# Autodesk Inventor assembly: Lift Assembly
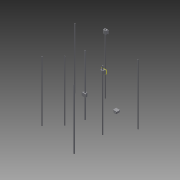
[picture p0: Inventor's stored thumbnail of the model, 180x180]
Saved by Autodesk Inventor 2013 (Build 170138000, 138)
## iProperties
Created: 2013-01-16
Part Number: Lift Assembly
Document SubType Name: Assembly
Designer: actoennies
Author: actoennies
## Documents named in this file (3)
- \\NNHSSRV2.hs.sd203.org\ACToennies$\Robotics\Lift\Lift Assembly.iam
- \\NNHSSRV2.hs.sd203.org\ACToennies$\Robotics\Lift\Tube.ipt
- \\NNHSSRV2.hs.sd203.org\ACToennies$\Inventor\Linear Bearing.ipt
## Components (12 placed, 2 different names)
1. Tube:1 — Mate:6, Mate:7
2. Tube:2 — Mate:1, Mate:2
3. Tube:3
4. Tube:4 — Mate:4, Mate:5
5. Tube:5
6. Tube:6
7. Tube:7
8. Tube:8
9. Linear Bearing:1 — Mate:1, Mate:2, Mate:3, Angle:1
10. Linear Bearing:2 — Mate:4, Mate:5
11. Linear Bearing:3 — Mate:6, Mate:7
12. Linear Bearing:4
## Relationships (8: Mate 7, Angle 1)
- Mate:1: Tube:2 ↔ Linear Bearing:1
- Mate:2: Tube:2 ↔ Linear Bearing:1
- Mate:3: Linear Bearing:1
- Angle:1 (0 deg): Linear Bearing:1
- Mate:4: Tube:4 ↔ Linear Bearing:2
- Mate:5: Tube:4 ↔ Linear Bearing:2
- Mate:6: Tube:1 ↔ Linear Bearing:3
- Mate:7: Tube:1 ↔ Linear Bearing:3
